# Autodesk Inventor assembly: ForeArm
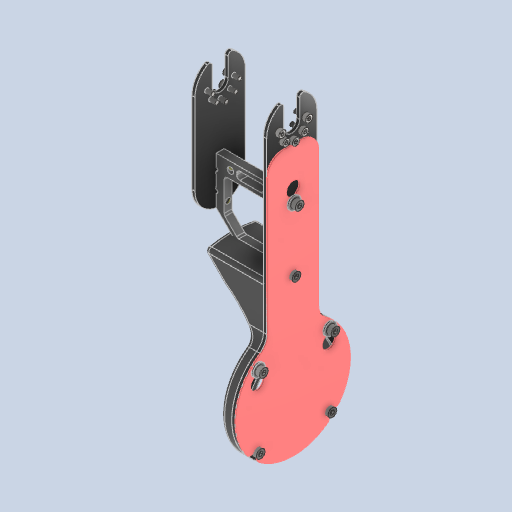
[picture p0: Inventor's stored thumbnail of the model, 512x512]
Saved by Autodesk Inventor 2022.3 (Build 263350000, 350)
## iProperties
Created: 2023-06-02
Part Number: ForeArm
Document SubType Name: Assembly
Designer: Masato Kubotera
Author: Masato Kubotera
## Documents named in this file (3)
- C:\Users\Masato\Desktop\SUSTAINA-OP\UpperBody\Arm\ForeArm.iam
- C:\Users\Masato\Desktop\SUSTAINA-OP\UpperBody\Arm\ForeArm_without_hand.iam
- C:\Users\Masato\Desktop\SUSTAINA-OP\UpperBody\Arm\ForeArm_hand.iam
## Components (2 placed, 2 different names)
1. ForeArm_without_hand:1 [sub-assembly] — Flush:1, Flush:2, Flush:3, Insert:1, Insert:2, Insert:3, Insert:4
2. ForeArm_hand:1 [sub-assembly] — Insert:1, Insert:2, Insert:3, Insert:4
## Relationships (7: Insert 4, Flush 3)
- Flush:1: ForeArm_without_hand:1
- Flush:2: ForeArm_without_hand:1
- Flush:3: ForeArm_without_hand:1
- Insert:1: ForeArm_without_hand:1 ↔ ForeArm_hand:1
- Insert:2: ForeArm_without_hand:1 ↔ ForeArm_hand:1
- Insert:3: ForeArm_without_hand:1 ↔ ForeArm_hand:1
- Insert:4: ForeArm_without_hand:1 ↔ ForeArm_hand:1
